# Autodesk Inventor assembly: claws_endeffector_7
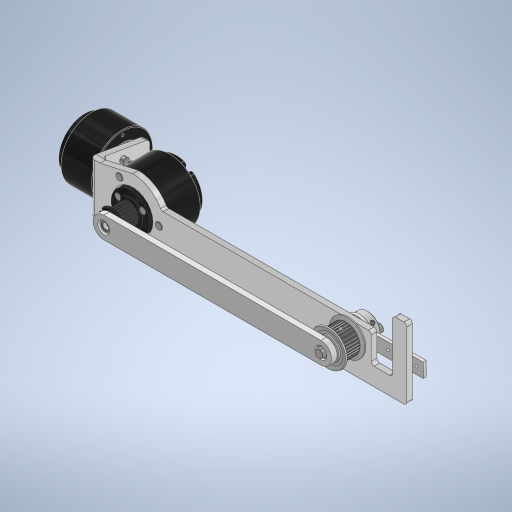
[picture p0: Inventor's stored thumbnail of the model, 512x512]
Saved by Autodesk Inventor 2024 (Build 280153000, 153)
## iProperties
Created: 2025-05-17
Part Number: claws_endeffector_7
Document SubType Name: Assembly
Designer: 1412z
Author: 1412z
## Documents named in this file (15)
- C:\Users\1412z\OneDrive\デスクトップ\rdclab\harvesting_robot\harvesting_endeffector\claws_endeffector\claws_endeffector_7.iam
- C:\Users\1412z\OneDrive\デスクトップ\rdclab\harvesting_robot\harvesting_endeffector\claws_endeffector\motor_holder\motor_holder_7.ipt
- C:\Users\1412z\OneDrive\デスクトップ\rdclab\harvesting_robot\harvesting_endeffector\claws_endeffector\GIM3505-08\GIM3505-8_with-driver.ipt
- C:\Users\1412z\OneDrive\デスクトップ\rdclab\harvesting_robot\harvesting_endeffector\claws_endeffector\misumi\HTPA22S2M100-A-V4-Z6-J3_Autodesk_Inventor_2024_20250304\HTPA22S2M100-A-V4-Z6-J3_0_a-3.ipt
- C:\Users\1412z\OneDrive\デスクトップ\rdclab\harvesting_robot\harvesting_endeffector\claws_endeffector\misumi\M2.5×4\M2.5×4.ipt
- C:\Users\1412z\OneDrive\デスクトップ\rdclab\harvesting_robot\harvesting_endeffector\claws_endeffector\misumi\SFL674ZZ_Autodesk_Inventor_2024_20250304\SFL674ZZ.ipt
- C:\Users\1412z\OneDrive\デスクトップ\rdclab\harvesting_robot\harvesting_endeffector\claws_endeffector\misumi\simring\simring_Φ4-Φ5.ipt
- C:\Users\1412z\OneDrive\デスクトップ\rdclab\harvesting_robot\harvesting_endeffector\claws_endeffector\misumi\HTPA32S2M100-A-P4_Autodesk_Inventor_2024_20250404\AIS2024\HTPA32S2M100-A-P4.iam
- C:\Users\1412z\OneDrive\デスクトップ\rdclab\harvesting_robot\harvesting_endeffector\claws_endeffector\misumi\washer\washer_M4.ipt
- C:\Users\1412z\OneDrive\デスクトップ\rdclab\harvesting_robot\harvesting_endeffector\claws_endeffector\motor_holder\motor_holder_top_2.ipt
- C:\Users\1412z\OneDrive\デスクトップ\rdclab\harvesting_robot\harvesting_endeffector\claws_endeffector\misumi\shaft\shaft_31.3mm.ipt
- C:\Users\1412z\OneDrive\デスクトップ\rdclab\harvesting_robot\harvesting_endeffector\claws_endeffector\cutter_part\cutter_board.ipt
- C:\Users\1412z\OneDrive\デスクトップ\rdclab\harvesting_robot\harvesting_endeffector\claws_endeffector\misumi\SSCMN4_Autodesk_Inventor_2024_20250310\AIS2024\SSCMN4.iam
- C:\Users\1412z\OneDrive\デスクトップ\rdclab\harvesting_robot\harvesting_endeffector\claws_endeffector\misumi\M3×4\M3×4.ipt
- C:\Users\1412z\OneDrive\デスクトップ\rdclab\harvesting_robot\harvesting_endeffector\claws_endeffector\misumi\M3×8\M3×8.ipt
## Components (29 placed, 14 different names)
1. motor_holder_7:1 — 回転:1, 回転:2, 回転:3, 回転:4, 回転:7, 回転:8, 回転:9, 回転:10, 回転:11, 回転:12, 回転:16, 回転:17
2. GIM3505-8_with-driver:1 — 回転:1, 回転:2, 回転:5, 回転:6
3. GIM3505-8_with-driver:2 — 回転:3, 回転:4
4. HTPA22S2M100-A-V4-Z6-J3_0_a-3:1 — 回転:5, 回転:6, 回転:13, 回転:14, 回転:15, 回転:21
5. M2.5×4:1 — 回転:9
6. M2.5×4:2 — 回転:12
7. M2.5×4:3 — 回転:11
8. M2.5×4:4 — 回転:10
9. M2.5×4:5 — 回転:8
10. M2.5×4:6 — 回転:7
11. M2.5×4:7 — 回転:13
12. M2.5×4:8 — 回転:14
13. M2.5×4:9 — 回転:15
14. SFL674ZZ:1 — 回転:16, 回転:19
15. SFL674ZZ:2 — 回転:17, 回転:18
16. simring_Φ4-Φ5:1 — 回転:19, 回転:27
17. simring_Φ4-Φ5:2 — 回転:18, 回転:20
18. HTPA32S2M100-A-P4:1 [sub-assembly] — 回転:20, 回転:22
19. washer_M4:1 — 回転:22, 回転:23
20. washer_M4:2 — 回転:21, 回転:24
21. motor_holder_top_2:1 — 回転:23, 回転:24, 回転:25, 回転:26
22. SFL674ZZ:3 — 回転:25, 回転:30
23. SFL674ZZ:4 — 回転:26
24. shaft_31.3mm:1 — 回転:30, 回転:31
25. cutter_board:1 — 回転:27, 回転:28, 回転:29
26. SSCMN4:1 [sub-assembly] — 回転:28, 回転:29, 回転:32, 回転:33
27. M3×4:1 — 回転:31
28. M3×8:1 — 回転:33
29. M3×8:2 — 回転:32
## Relationships (33: RevoluteJoint 33)
- 回転:1 [RevoluteJoint]: motor_holder_7:1 ↔ GIM3505-8_with-driver:1
- 回転:2 [RevoluteJoint]: motor_holder_7:1 ↔ GIM3505-8_with-driver:1
- 回転:3 [RevoluteJoint]: motor_holder_7:1 ↔ GIM3505-8_with-driver:2
- 回転:4 [RevoluteJoint]: motor_holder_7:1 ↔ GIM3505-8_with-driver:2
- 回転:5 [RevoluteJoint]: GIM3505-8_with-driver:1 ↔ HTPA22S2M100-A-V4-Z6-J3_0_a-3:1
- 回転:6 [RevoluteJoint]: GIM3505-8_with-driver:1 ↔ HTPA22S2M100-A-V4-Z6-J3_0_a-3:1
- 回転:7 [RevoluteJoint]: motor_holder_7:1 ↔ M2.5×4:6
- 回転:8 [RevoluteJoint]: motor_holder_7:1 ↔ M2.5×4:5
- 回転:9 [RevoluteJoint]: motor_holder_7:1 ↔ M2.5×4:1
- 回転:10 [RevoluteJoint]: motor_holder_7:1 ↔ M2.5×4:4
- 回転:11 [RevoluteJoint]: motor_holder_7:1 ↔ M2.5×4:3
- 回転:12 [RevoluteJoint]: motor_holder_7:1 ↔ M2.5×4:2
- 回転:13 [RevoluteJoint]: HTPA22S2M100-A-V4-Z6-J3_0_a-3:1 ↔ M2.5×4:7
- 回転:14 [RevoluteJoint]: HTPA22S2M100-A-V4-Z6-J3_0_a-3:1 ↔ M2.5×4:8
- 回転:15 [RevoluteJoint]: HTPA22S2M100-A-V4-Z6-J3_0_a-3:1 ↔ M2.5×4:9
- 回転:16 [RevoluteJoint]: motor_holder_7:1 ↔ SFL674ZZ:1
- 回転:17 [RevoluteJoint]: motor_holder_7:1 ↔ SFL674ZZ:2
- 回転:18 [RevoluteJoint]: SFL674ZZ:2 ↔ simring_Φ4-Φ5:2
- 回転:19 [RevoluteJoint]: SFL674ZZ:1 ↔ simring_Φ4-Φ5:1
- 回転:20 [RevoluteJoint]: simring_Φ4-Φ5:2 ↔ HTPA32S2M100-A-P4:1
- 回転:21 [RevoluteJoint]: HTPA22S2M100-A-V4-Z6-J3_0_a-3:1 ↔ washer_M4:2
- 回転:22 [RevoluteJoint]: HTPA32S2M100-A-P4:1 ↔ washer_M4:1
- 回転:23 [RevoluteJoint]: washer_M4:1 ↔ motor_holder_top_2:1
- 回転:24 [RevoluteJoint]: washer_M4:2 ↔ motor_holder_top_2:1
- 回転:25 [RevoluteJoint]: motor_holder_top_2:1 ↔ SFL674ZZ:3
- 回転:26 [RevoluteJoint]: motor_holder_top_2:1 ↔ SFL674ZZ:4
- 回転:27 [RevoluteJoint]: simring_Φ4-Φ5:1 ↔ cutter_board:1
- 回転:28 [RevoluteJoint]: cutter_board:1 ↔ SSCMN4:1
- 回転:29 [RevoluteJoint]: cutter_board:1 ↔ SSCMN4:1
- 回転:30 [RevoluteJoint]: SFL674ZZ:3 ↔ shaft_31.3mm:1
- 回転:31 [RevoluteJoint]: shaft_31.3mm:1 ↔ M3×4:1
- 回転:32 [RevoluteJoint]: SSCMN4:1 ↔ M3×8:2
- 回転:33 [RevoluteJoint]: SSCMN4:1 ↔ M3×8:1
